# Autodesk Inventor assembly: total
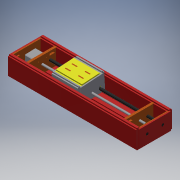
[picture p0: Inventor's stored thumbnail of the model, 180x180]
Saved by Autodesk Inventor 2017 (Build 210142000, 142)
## iProperties
Created: 2015-10-11
Part Number: total
Document SubType Name: Assembly
Designer: daniel
Author: daniel
## Documents named in this file (5)
- C:\Users\daniel\Documents\GitHub\cardboard-stage-metric\stage\total.iam
- C:\Users\daniel\Documents\GitHub\cardboard-stage-metric\stage\a.iam
- C:\Users\daniel\Documents\GitHub\cardboard-stage-metric\stage\carriage.iam
- C:\Users\daniel\Documents\GitHub\cardboard-stage-metric\stage\shaft.ipt
- C:\Users\daniel\Documents\GitHub\cardboard-stage-metric\stage\inner.iam
## Components (5 placed, 4 different names)
1. a:1 [sub-assembly] — Insert:1, Insert:2, Flush:1, Flush:2, Flush:3, Mate:1, Mate:2, Mate:3
2. carriage:1 [sub-assembly] — Cylindrical:2
3. shaft:1 — Insert:1
4. shaft:2 — Insert:2, Cylindrical:2
5. inner:1 [sub-assembly] — Mate:1, Mate:2, Mate:3
## Relationships (9: Flush 3, Mate 3, Insert 2, CylindricalJoint 1)
- Insert:1: a:1 ↔ shaft:1
- Insert:2: a:1 ↔ shaft:2
- Flush:1: a:1
- Flush:2: a:1
- Flush:3: a:1
- Mate:1: a:1 ↔ inner:1
- Mate:2: a:1 ↔ inner:1
- Mate:3: a:1 ↔ inner:1
- Cylindrical:2: carriage:1 ↔ shaft:2
